# Autodesk Inventor assembly: leg
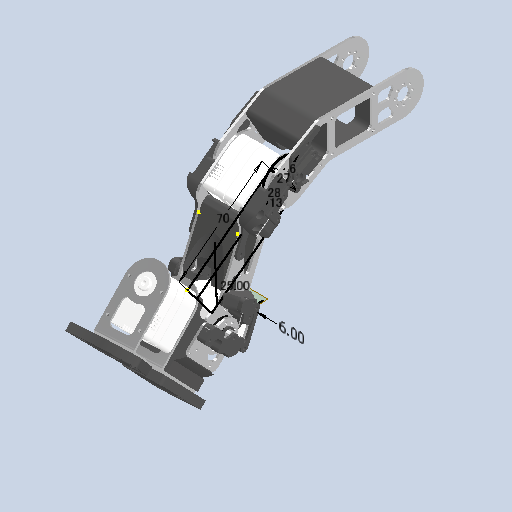
[picture p0: Inventor's stored thumbnail of the model, 512x512]
Saved by Autodesk Inventor 2024.1 (Build 281209000, 209)
## iProperties
Created: 2024-02-11
Part Number: leg
Document SubType Name: Assembly
Designer: hibik
Author: hibik
## Documents named in this file (21)
- C:\Users\hibik\Documents\Robomech\HR\Eglantyne\hard\leg\leg.iam
- C:\Users\hibik\Documents\Robomech\HR\Eglantyne\hard\leg\leg_under.iam
- C:\Users\hibik\Documents\Robomech\HR\Eglantyne\hard\leg\leg_upper.iam
- C:\Users\hibik\Documents\Robomech\HR\Eglantyne\hard\leg\toe.iam
- C:\Users\hibik\Desktop\ロボメカ\HR\2024.02.11 Rl\spring_180,90.ipt
- C:\Users\hibik\Documents\Robomech\HR\Eglantyne\hard\leg\leg_springjoint_bace_left.ipt
- C:\Users\hibik\Documents\Robomech\HR\Eglantyne\hard\leg\leg_springjoint_cover_left.ipt
- C:\Users\hibik\Documents\Robomech\HR\Eglantyne\hard\leg\leg_springjoint_bace_under_left.ipt
- C:\Users\hibik\Documents\Robomech\HR\Eglantyne\hard\leg\leg_springjoint_cover_under_left.ipt
- C:\Users\hibik\Documents\Robomech\HR\Eglantyne\hard\leg\toe_springjoint_bace_under_left.ipt
- C:\Users\hibik\Documents\Robomech\HR\Eglantyne\hard\leg\toe_springjoint_bace_upper_left.ipt
- C:\Users\hibik\Documents\Robomech\HR\Eglantyne\hard\leg\toe_springjoint_cover_under_left.ipt
- C:\Users\hibik\Documents\Robomech\HR\Eglantyne\hard\leg\toe_springjoint_cover_upper_left.ipt
- C:\Users\hibik\Documents\Robomech\HR\Eglantyne\hard\leg\leg_springjoint_bace_right.ipt
- C:\Users\hibik\Documents\Robomech\HR\Eglantyne\hard\leg\leg_springjoint_bace_under_right.ipt
- C:\Users\hibik\Documents\Robomech\HR\Eglantyne\hard\leg\leg_springjoint_cover_right.ipt
- C:\Users\hibik\Documents\Robomech\HR\Eglantyne\hard\leg\leg_springjoint_cover_under_right.ipt
- C:\Users\hibik\Documents\Robomech\HR\Eglantyne\hard\leg\toe_springjoint_bace_under_right.ipt
- C:\Users\hibik\Documents\Robomech\HR\Eglantyne\hard\leg\toe_springjoint_bace_upper_right.ipt
- C:\Users\hibik\Documents\Robomech\HR\Eglantyne\hard\leg\toe_springjoint_cover_under_right.ipt
- C:\Users\hibik\Documents\Robomech\HR\Eglantyne\hard\leg\toe_springjoint_cover_upper_right.ipt
## Components (27 placed, 20 different names)
1. leg_under:1 [sub-assembly] — 挿入:1, 挿入:2, メイト:1, フラッシュ:1, 挿入:12, 挿入:18, フラッシュ:2, 挿入:25, 挿入:26, 挿入:36, 挿入:37
2. leg_upper:1 [sub-assembly] — 挿入:1, 挿入:13, 挿入:27, 挿入:28
3. toe:1 [sub-assembly] — 挿入:2, 挿入:16, 挿入:17, 挿入:40, 挿入:41
4. spring_180,90:1 — 挿入:3, メイト:2
5. spring_180,90:2 — 挿入:3, 角度:1
6. leg_springjoint_cover_under_left:1 — 挿入:10, 挿入:11
7. leg_springjoint_bace_under_left:1 — メイト:1, フラッシュ:1, 挿入:10, 挿入:11, 挿入:12, メイト:2
8. leg_springjoint_bace_left:1 — 挿入:13, 角度:1, 挿入:14, 挿入:15
9. leg_springjoint_cover_left:1 — 挿入:14, 挿入:15
10. toe_springjoint_bace_under_left:1 — 挿入:16, 挿入:17, 挿入:19, 正接:1, 挿入:23, 角度:2
11. toe_springjoint_bace_upper_left:1 — 挿入:18, フラッシュ:2, 挿入:20, 挿入:21, 挿入:22, 角度:3
12. toe_springjoint_cover_under_left:1 — 挿入:19, 正接:1
13. toe_springjoint_cover_upper_left:1 — 挿入:20, 挿入:21, 挿入:22
14. spring_180,90:3 — 挿入:23, 挿入:24, 角度:2
15. spring_180,90:4 — 挿入:24, 角度:3
16. leg_springjoint_bace_right:1 — 挿入:27, 挿入:28, 挿入:29, 挿入:30, 挿入:35, 角度:4
17. leg_springjoint_bace_under_right:1 — 挿入:25, 挿入:26, 挿入:31, 挿入:32, 角度:5
18. leg_springjoint_cover_right:1 — 挿入:29, 挿入:30
19. leg_springjoint_cover_under_right:1 — 挿入:31, 挿入:32
20. spring_180,90:5 — 挿入:33, 角度:4
21. spring_180,90:6 — 挿入:33, 挿入:35, 角度:5
22. toe_springjoint_bace_under_right:1 — 挿入:40, 挿入:41, 挿入:42, 挿入:43, 挿入:45, 角度:6
23. toe_springjoint_bace_upper_right:1 — 挿入:36, 挿入:37, 挿入:38, 挿入:39, 角度:7
24. toe_springjoint_cover_under_right:1 — 挿入:42, 挿入:43
25. toe_springjoint_cover_upper_right:1 — 挿入:38, 挿入:39
26. spring_180,90:7 — 挿入:44, 挿入:45, 角度:7
27. spring_180,90:8 — 挿入:44, 角度:6
## Relationships (50: Insert 38, Angle 7, Mate 2, Flush 2, Tangent 1)
- 挿入:1 [Insert]: leg_under:1 ↔ leg_upper:1
- 挿入:2 [Insert]: leg_under:1 ↔ toe:1
- 挿入:3 [Insert]: spring_180,90:1 ↔ spring_180,90:2
- メイト:1 [Mate]: leg_under:1 ↔ leg_springjoint_bace_under_left:1
- フラッシュ:1 [Flush]: leg_under:1 ↔ leg_springjoint_bace_under_left:1
- 挿入:10 [Insert]: leg_springjoint_cover_under_left:1 ↔ leg_springjoint_bace_under_left:1
- 挿入:11 [Insert]: leg_springjoint_cover_under_left:1 ↔ leg_springjoint_bace_under_left:1
- 挿入:12 [Insert]: leg_under:1 ↔ leg_springjoint_bace_under_left:1
- メイト:2 [Mate] (0.5 mm): spring_180,90:1 ↔ leg_springjoint_bace_under_left:1
- 挿入:13 [Insert]: leg_upper:1 ↔ leg_springjoint_bace_left:1
- 角度:1 [Angle] (180 deg): spring_180,90:2 ↔ leg_springjoint_bace_left:1
- 挿入:14 [Insert]: leg_springjoint_bace_left:1 ↔ leg_springjoint_cover_left:1
- 挿入:15 [Insert]: leg_springjoint_bace_left:1 ↔ leg_springjoint_cover_left:1
- 挿入:16 [Insert]: toe:1 ↔ toe_springjoint_bace_under_left:1
- 挿入:17 [Insert]: toe:1 ↔ toe_springjoint_bace_under_left:1
- 挿入:18 [Insert]: leg_under:1 ↔ toe_springjoint_bace_upper_left:1
- フラッシュ:2 [Flush]: leg_under:1 ↔ toe_springjoint_bace_upper_left:1
- 挿入:19 [Insert]: toe_springjoint_bace_under_left:1 ↔ toe_springjoint_cover_under_left:1
- 正接:1 [Tangent]: toe_springjoint_bace_under_left:1 ↔ toe_springjoint_cover_under_left:1
- 挿入:20 [Insert]: toe_springjoint_bace_upper_left:1 ↔ toe_springjoint_cover_upper_left:1
- 挿入:21 [Insert]: toe_springjoint_bace_upper_left:1 ↔ toe_springjoint_cover_upper_left:1
- 挿入:22 [Insert]: toe_springjoint_bace_upper_left:1 ↔ toe_springjoint_cover_upper_left:1
- 挿入:23 [Insert]: toe_springjoint_bace_under_left:1 ↔ spring_180,90:3
- 挿入:24 [Insert]: spring_180,90:3 ↔ spring_180,90:4
- 角度:2 [Angle] (180 deg): toe_springjoint_bace_under_left:1 ↔ spring_180,90:3
- 角度:3 [Angle] (180 deg): toe_springjoint_bace_upper_left:1 ↔ spring_180,90:4
- 挿入:25 [Insert]: leg_under:1 ↔ leg_springjoint_bace_under_right:1
- 挿入:26 [Insert]: leg_under:1 ↔ leg_springjoint_bace_under_right:1
- 挿入:27 [Insert]: leg_upper:1 ↔ leg_springjoint_bace_right:1
- 挿入:28 [Insert]: leg_upper:1 ↔ leg_springjoint_bace_right:1
- 挿入:29 [Insert]: leg_springjoint_bace_right:1 ↔ leg_springjoint_cover_right:1
- 挿入:30 [Insert]: leg_springjoint_bace_right:1 ↔ leg_springjoint_cover_right:1
- 挿入:31 [Insert]: leg_springjoint_bace_under_right:1 ↔ leg_springjoint_cover_under_right:1
- 挿入:32 [Insert]: leg_springjoint_bace_under_right:1 ↔ leg_springjoint_cover_under_right:1
- 挿入:33 [Insert]: spring_180,90:5 ↔ spring_180,90:6
- 挿入:35 [Insert]: leg_springjoint_bace_right:1 ↔ spring_180,90:6
- 角度:4 [Angle] (180 deg): leg_springjoint_bace_right:1 ↔ spring_180,90:5
- 角度:5 [Angle] (180 deg): leg_springjoint_bace_under_right:1 ↔ spring_180,90:6
- 挿入:36 [Insert]: leg_under:1 ↔ toe_springjoint_bace_upper_right:1
- 挿入:37 [Insert]: leg_under:1 ↔ toe_springjoint_bace_upper_right:1
- 挿入:38 [Insert]: toe_springjoint_bace_upper_right:1 ↔ toe_springjoint_cover_upper_right:1
- 挿入:39 [Insert]: toe_springjoint_bace_upper_right:1 ↔ toe_springjoint_cover_upper_right:1
- 挿入:40 [Insert]: toe:1 ↔ toe_springjoint_bace_under_right:1
- 挿入:41 [Insert]: toe:1 ↔ toe_springjoint_bace_under_right:1
- 挿入:42 [Insert]: toe_springjoint_bace_under_right:1 ↔ toe_springjoint_cover_under_right:1
- 挿入:43 [Insert]: toe_springjoint_bace_under_right:1 ↔ toe_springjoint_cover_under_right:1
- 挿入:44 [Insert]: spring_180,90:7 ↔ spring_180,90:8
- 挿入:45 [Insert]: toe_springjoint_bace_under_right:1 ↔ spring_180,90:7
- 角度:6 [Angle] (180 deg): toe_springjoint_bace_under_right:1 ↔ spring_180,90:8
- 角度:7 [Angle] (180 deg): toe_springjoint_bace_upper_right:1 ↔ spring_180,90:7
